# Autodesk Inventor assembly: Assembly1
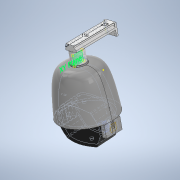
[picture p0: Inventor's stored thumbnail of the model, 180x180]
Saved by Autodesk Inventor 2021.1 (Build 251245010, 245A)
## iProperties
Created: 2023-07-02
Part Number: Assembly1
Document SubType Name: Assembly
Designer: Drake
Author: Drake
## Documents named in this file (7)
- C:\bkp\FYPDESIGN1\Assembly1.iam
- C:\bkp\FYPDESIGN1\TopBracket.ipt
- C:\bkp\FYPDESIGN1\Motor.ipt
- C:\bkp\FYPDESIGN1\EnclosingRevolver.ipt
- C:\bkp\FYPDESIGN1\CameraHolder2.ipt
- C:\bkp\FYPDESIGN1\SG90_Model_B.ipt
- C:\bkp\FYPDESIGN1\sg90CustomArm.ipt
## Components (6 placed, 6 different names)
1. TopBracket:1 — Mate:1, Mate:2, Mate:4, Rigid:2
2. Motor:3 — Mate:1, Mate:2
3. EnclosingRevolver:1 — Rigid:2, Mate:3, Mate:4, Mate:7
4. CameraHolder2:1 — Mate:3, Mate:5, Mate:6, Insert:1
5. SG90_Model_B:1 — Mate:5, Mate:6, Insert:1, Rotation:1
6. sg90CustomArm:1 — Mate:7, Rotation:1
## Relationships (10: Mate 7, WeldJoint 1, Insert 1, RelateRotation 1)
- Mate:1: TopBracket:1 ↔ Motor:3
- Mate:2: TopBracket:1 ↔ Motor:3
- Rigid:2 [WeldJoint] (-2.54 mm): TopBracket:1 ↔ EnclosingRevolver:1
- Mate:3: EnclosingRevolver:1 ↔ CameraHolder2:1
- Mate:4: TopBracket:1 ↔ EnclosingRevolver:1
- Mate:5: CameraHolder2:1 ↔ SG90_Model_B:1
- Mate:6: CameraHolder2:1 ↔ SG90_Model_B:1
- Insert:1: CameraHolder2:1 ↔ SG90_Model_B:1
- Mate:7: EnclosingRevolver:1 ↔ sg90CustomArm:1
- Rotation:1 [RelateRotation] (1 ul): SG90_Model_B:1 ↔ sg90CustomArm:1
